# Autodesk Inventor assembly: WristDifferential
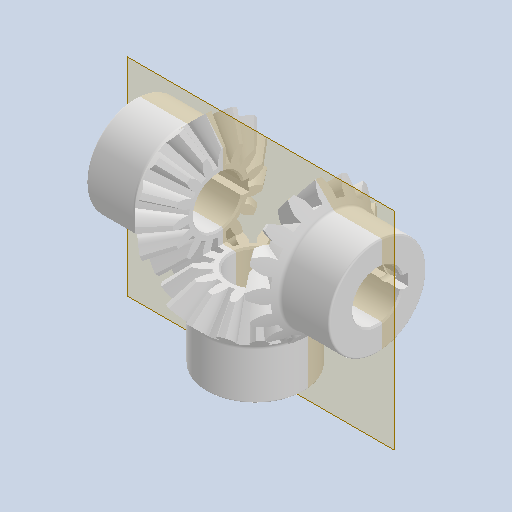
[picture p0: Inventor's stored thumbnail of the model, 512x512]
Saved by Autodesk Inventor 2025.1 (Build 291241020, 241B)
## iProperties
Created: 2023-11-15
Part Number: WristDifferential
Document SubType Name: Assembly
Designer: megan
Author: megan
## Documents named in this file (2)
- C:\Users\t205b\OneDrive\Documents\Github\BehrendURCMechanical\CAD\Chassis V3\Wrist\WristDifferential.iam
- C:\Users\t205b\OneDrive\Documents\Github\BehrendURCMechanical\CAD\Chassis V3\Wrist\6843K13_Metal Miter Gear.ipt
## Components (3 placed, 1 different names)
1. 6843K13_Metal Miter Gear:1 — Mate:3
2. 6843K13_Metal Miter Gear:2 — Mate:1, Mate:2
3. 6843K13_Metal Miter Gear:3 — Mate:1
## Relationships (3: Mate 3)
- Mate:1: 6843K13_Metal Miter Gear:2 ↔ 6843K13_Metal Miter Gear:3
- Mate:2: 6843K13_Metal Miter Gear:2
- Mate:3: 6843K13_Metal Miter Gear:1
